# Autodesk Inventor assembly: エンコーダ取り付け
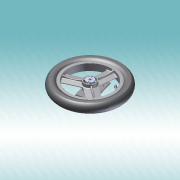
[picture p0: Inventor's stored thumbnail of the model, 180x180]
Saved by Autodesk Inventor 2015 (Build 190159000, 159)
## iProperties
Created: 2016-02-18
Part Number: エンコーダ取り付け
Document SubType Name: Assembly
Designer: buzztaka
Author: buzztaka
## Documents named in this file (10)
- C:\Users\buzztaka\Documents\tukuba\i-cart-middle_3d-model\計測輪アセンブル\エンコーダ取り付け ver2.iam
- C:\Users\buzztaka\Documents\tukuba\i-cart-middle_3d-model\計測輪アセンブル\meh-30-pエンコーダ.ipt
- C:\Users\buzztaka\Documents\tukuba\i-cart-middle_3d-model\計測輪アセンブル\wheel_12inch.ipt
- C:\Users\buzztaka\Documents\tukuba\i-cart-middle_3d-model\計測輪アセンブル\wheel-hub.ipt
- C:\Users\buzztaka\Documents\tukuba\i-cart-middle_3d-model\計測輪アセンブル\whelelcapholl.ipt
- C:\Users\buzztaka\Documents\tukuba\i-cart-middle_3d-model\計測輪アセンブル\スプリングフランジ用ワッシャー（座金）.ipt
- C:\Users\buzztaka\Documents\tukuba\i-cart-middle_3d-model\計測輪アセンブル\スプリングフランジ0.1mm.ipt
- C:\Users\buzztaka\Documents\tukuba\i-cart-middle_3d-model\計測輪アセンブル\計測輪シャフトver1.ipt
- C:\Users\buzztaka\Documents\tukuba\i-cart-middle_3d-model\計測輪アセンブル\エンコーダ取り付け板.ipt
- C:\Users\buzztaka\Documents\Inventor\Content Center Files\R2015\ja-JP\JIS B 1181 R C (2)\JIS B 1181 - M10(9).ipt
## Components (11 placed, 9 different names)
1. wheel_12inch:1 — 挿入:7, 挿入:8, 挿入:9, 挿入:10
2. wheel-hub:1 — 挿入:7, 挿入:8
3. whelelcapholl:1 — 挿入:9, 挿入:10, 挿入:18
4. meh-30-pエンコーダ:1 — 挿入:11, 挿入:12, 挿入:13, 挿入:16
5. スプリングフランジ用ワッシャー（座金）:1 — 挿入:12
6. スプリングフランジ用ワッシャー（座金）:2 — 挿入:11, 挿入:14
7. スプリングフランジ用ワッシャー（座金）:3 — 挿入:13, 挿入:15
8. スプリングフランジ0.1mm:1 — 挿入:14, 挿入:15, 挿入:17
9. 計測輪シャフトver1:1 — 挿入:16, 挿入:18, 挿入:19
10. エンコーダ取り付け板:1 — 挿入:17
11. JIS B 1181 仕上程度 並 等級 2 - メートル 等級 2 仕上程度 並 M10:1 — 挿入:19
## Relationships (13: Insert 13)
- 挿入:7 [Insert]: wheel_12inch:1 ↔ wheel-hub:1
- 挿入:8 [Insert]: wheel_12inch:1 ↔ wheel-hub:1
- 挿入:9 [Insert]: wheel_12inch:1 ↔ whelelcapholl:1
- 挿入:10 [Insert]: wheel_12inch:1 ↔ whelelcapholl:1
- 挿入:11 [Insert]: meh-30-pエンコーダ:1 ↔ スプリングフランジ用ワッシャー（座金）:2
- 挿入:12 [Insert]: meh-30-pエンコーダ:1 ↔ スプリングフランジ用ワッシャー（座金）:1
- 挿入:13 [Insert]: meh-30-pエンコーダ:1 ↔ スプリングフランジ用ワッシャー（座金）:3
- 挿入:14 [Insert]: スプリングフランジ用ワッシャー（座金）:2 ↔ スプリングフランジ0.1mm:1
- 挿入:15 [Insert]: スプリングフランジ用ワッシャー（座金）:3 ↔ スプリングフランジ0.1mm:1
- 挿入:16 [Insert] (-10 mm): meh-30-pエンコーダ:1 ↔ 計測輪シャフトver1:1
- 挿入:17 [Insert]: スプリングフランジ0.1mm:1 ↔ エンコーダ取り付け板:1
- 挿入:18 [Insert]: whelelcapholl:1 ↔ 計測輪シャフトver1:1
- 挿入:19 [Insert] (2 mm): 計測輪シャフトver1:1 ↔ JIS B 1181 仕上程度 並 等級 2 - メートル 等級 2 仕上程度 並 M10:1
